# Autodesk Inventor assembly: Belastungstest
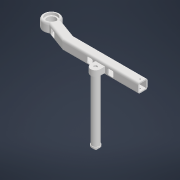
[picture p0: Inventor's stored thumbnail of the model, 180x180]
Saved by Autodesk Inventor 2021 (Build 250183000, 183)
## iProperties
Created: 2021-03-06
Part Number: Belastungstest
Document SubType Name: Assembly
Designer: Ctroi
Author: Ctroi
## Documents named in this file (15)
- G:\Roverprojekt\Github Projekt\Rover\Belastungstest.iam
- G:\Roverprojekt\Github Projekt\Rover\Verbindung_Rocker_Body.ipt
- G:\Roverprojekt\Github Projekt\Rover\Rocker_hinten.ipt
- G:\Roverprojekt\Github Projekt\Rover\Belastungstest\AIP\FEA\djd71v0qo.fins
- G:\Roverprojekt\Github Projekt\Rover\Belastungstest\AIP\FEA\djd71v0qo.fsat
- G:\Roverprojekt\Github Projekt\Rover\Belastungstest\AIP\FEA\djd71v0qo.ftes
- G:\Roverprojekt\Github Projekt\Rover\Belastungstest\AIP\FEA\djd71v0qo.fwiz
- G:\Roverprojekt\Github Projekt\Rover\Belastungstest\AIP\FEA\djd71v0qp.fins
- G:\Roverprojekt\Github Projekt\Rover\Belastungstest\AIP\FEA\djd71v0qp.fsat
- G:\Roverprojekt\Github Projekt\Rover\Belastungstest\AIP\FEA\djd71v0qp.ftes
- G:\Roverprojekt\Github Projekt\Rover\Belastungstest\AIP\FEA\djd71v0qp.fwiz
- G:\Roverprojekt\Github Projekt\Rover\Belastungstest\AIP\FEA\djd71v0sg.fmsh
- G:\Roverprojekt\Github Projekt\Rover\Belastungstest\AIP\FEA\djd71v0sh.fres
- G:\Roverprojekt\Github Projekt\Rover\Belastungstest\AIP\FEA\djd71v0u8.fmsh
- G:\Roverprojekt\Github Projekt\Rover\Belastungstest\AIP\FEA\djd71v0u9.fres
## Components (2 placed, 2 different names)
1. Verbindung_Rocker_Body:1 — Passend:3
2. Fahrwerk_rocker_hinten:1 — Passend:3
## Relationships (1: Mate 1)
- Passend:3 [Mate]: Verbindung_Rocker_Body:1 ↔ Fahrwerk_rocker_hinten:1
## Named parameters: sa_0 = 2000, sa_1 = 2000
note: some values were not read from the file. Shown as the stored number, unit unknown: "sa_0", "sa_1".
